# Autodesk Inventor assembly: Overview
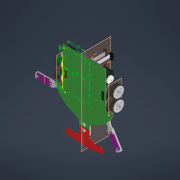
[picture p0: Inventor's stored thumbnail of the model, 180x180]
Saved by Autodesk Inventor 2022 (Build 260153000, 153)
## iProperties
Created: 2021-10-05
Part Number: Overview
Document SubType Name: Assembly
Designer: shiok
Mass: 71.5322 g
Surface Area: 774.809 cm^2
Volume: 60.689 cm^3
Density: 1.17867 g/cm^3
Author: shiok
## Documents named in this file (11)
- C:\Users\shiok\Documents\GitHub\murakumo\inventor\Overview.iam
- C:\Users\shiok\Documents\GitHub\murakumo\inventor\flame.ipt
- C:\Users\shiok\Documents\GitHub\murakumo\inventor\Motor.iam
- C:\Users\shiok\Documents\GitHub\murakumo\inventor\Motor_MIR1.iam
- C:\Users\shiok\Documents\GitHub\murakumo\inventor\sensor.ipt
- C:\Users\shiok\Documents\GitHub\murakumo\inventor\SideSensorCircuit.ipt
- C:\Users\shiok\Documents\GitHub\murakumo\inventor\top.ipt
- C:\Users\shiok\Documents\GitHub\murakumo\inventor\jump.ipt
- C:\Users\shiok\Documents\GitHub\murakumo\inventor\SideSensorMount.ipt
- C:\Users\shiok\Documents\GitHub\murakumo\inventor\SideSensorCircuit_MIR3.ipt
- C:\Users\shiok\Documents\GitHub\murakumo\inventor\SideSensorMount_MIR.ipt
## Components (10 placed, 10 different names)
1. flame:1 — フラッシュ:1, フラッシュ:2, フラッシュ:3, 挿入:17, メイト:10, メイト:15, フラッシュ:7, メイト:16, 挿入:21, メイト:20, 挿入:25, メイト:22
2. Motor:1 [sub-assembly] — 対称度:2, メイト:10, 対称度:3, 挿入:21, 挿入:24
3. sensor:1 — フラッシュ:6, メイト:15, フラッシュ:7, メイト:17, メイト:18
4. Motor_MIR1:1 [sub-assembly] — 挿入:17, 対称度:2, 対称度:3, メイト:12, メイト:13, メイト:14, 挿入:28
5. top:1 — メイト:12, メイト:13, メイト:14
6. jump:1 — メイト:16, メイト:17, メイト:18
7. SideSensorCircuit:1 — メイト:19, フラッシュ:8, 挿入:22, 挿入:23
8. SideSensorMount:1 — メイト:19, フラッシュ:8, 挿入:22, 挿入:23, 挿入:24, メイト:20, 挿入:25
9. SideSensorCircuit_MIR3:1 — 挿入:26, 挿入:27, フラッシュ:9, メイト:21
10. SideSensorMount_MIR:1 — 挿入:26, 挿入:27, フラッシュ:9, メイト:21, 挿入:28, メイト:22
## Relationships (30: Mate 12, Insert 9, Flush 7, Symmetry 2)
- フラッシュ:1 [Flush]: flame:1
- フラッシュ:2 [Flush]: flame:1
- フラッシュ:3 [Flush]: flame:1
- フラッシュ:6 [Flush]: sensor:1
- 挿入:17 [Insert]: flame:1 ↔ Motor_MIR1:1
- 対称度:2 [Symmetry]: Motor:1 ↔ Motor_MIR1:1
- メイト:10 [Mate]: flame:1 ↔ Motor:1
- 対称度:3 [Symmetry]: Motor:1 ↔ Motor_MIR1:1
- メイト:12 [Mate]: Motor_MIR1:1 ↔ top:1
- メイト:13 [Mate]: Motor_MIR1:1 ↔ top:1
- メイト:14 [Mate]: Motor_MIR1:1 ↔ top:1
- メイト:15 [Mate]: flame:1 ↔ sensor:1
- フラッシュ:7 [Flush]: flame:1 ↔ sensor:1
- メイト:16 [Mate]: flame:1 ↔ jump:1
- メイト:17 [Mate]: sensor:1 ↔ jump:1
- メイト:18 [Mate]: sensor:1 ↔ jump:1
- 挿入:21 [Insert]: flame:1 ↔ Motor:1
- メイト:19 [Mate]: SideSensorCircuit:1 ↔ SideSensorMount:1
- フラッシュ:8 [Flush]: SideSensorCircuit:1 ↔ SideSensorMount:1
- 挿入:22 [Insert]: SideSensorCircuit:1 ↔ SideSensorMount:1
- 挿入:23 [Insert]: SideSensorCircuit:1 ↔ SideSensorMount:1
- 挿入:24 [Insert]: Motor:1 ↔ SideSensorMount:1
- メイト:20 [Mate]: flame:1 ↔ SideSensorMount:1
- 挿入:25 [Insert]: flame:1 ↔ SideSensorMount:1
- 挿入:26 [Insert]: SideSensorCircuit_MIR3:1 ↔ SideSensorMount_MIR:1
- 挿入:27 [Insert]: SideSensorCircuit_MIR3:1 ↔ SideSensorMount_MIR:1
- フラッシュ:9 [Flush]: SideSensorCircuit_MIR3:1 ↔ SideSensorMount_MIR:1
- メイト:21 [Mate]: SideSensorCircuit_MIR3:1 ↔ SideSensorMount_MIR:1
- 挿入:28 [Insert]: Motor_MIR1:1 ↔ SideSensorMount_MIR:1
- メイト:22 [Mate]: flame:1 ↔ SideSensorMount_MIR:1
